# Autodesk Inventor assembly: minimal_frame_assembly
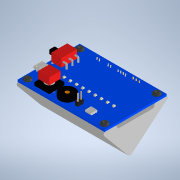
[picture p0: Inventor's stored thumbnail of the model, 180x180]
Saved by Autodesk Inventor 2020 (Build 240168000, 168)
## iProperties
Created: 2020-07-05
Part Number: minimal_frame_assembly
Document SubType Name: Assembly
Designer: Lukasz
Author: Lukasz
## Documents named in this file (7)
- C:\LUKE\PROJECTS\POMODORO\Mechanical\Assemblies\minimal_frame_assembly.iam
- C:\LUKE\PROJECTS\POMODORO\Mechanical\Assemblies\Board\Board_Pomodoro_v1.0.iam
- C:\LUKE\PROJECTS\POMODORO\Mechanical\Parts\minimal_frame_right.ipt
- C:\LUKE\PROJECTS\POMODORO\Mechanical\Parts\Standard\knurled_insert_M3_4.ipt
- C:\LUKE\PROJECTS\POMODORO\Mechanical\Parts\Standard\BATTERY_1S_560MAH_AKYGA.ipt
- C:\Users\Lukasz\Documents\Inventor\Content Center Files\R2020\en-US\ISO 7380-1\ISO 7380-1 - M3 x 6.ipt
- C:\LUKE\PROJECTS\POMODORO\Mechanical\Parts\battery_mount_1s_500mah.ipt
## Components (10 placed, 6 different names)
1. Board_Pomodoro_v1.0:1 [sub-assembly] — Rotational:1, Rotational:2, Flush:1, Angle:1, Rigid:3, Rigid:4, Rigid:5, Rigid:6
2. minimal_frame_right:1 — Rotational:1, Rotational:2, Rigid:1, Rigid:2, Mate:1, Cylindrical:1, Cylindrical:2
3. knurled_insert_M3_4:1 — Rigid:2
4. knurled_insert_M3_4:2 — Rigid:1
5. BATTERY_1S_560MAH_AKYGA:1 — Flush:1, Angle:1, Mate:1, Mate:2, Mate:3
6. ISO 7380-1 M3 x 6:1 — Rigid:3
7. ISO 7380-1 M3 x 6:2 — Rigid:6
8. ISO 7380-1 M3 x 6:3 — Rigid:4
9. ISO 7380-1 M3 x 6:4 — Rigid:5
10. battery_mount_1s_500mah:2 — Mate:2, Mate:3, Cylindrical:1, Cylindrical:2
## Relationships (15: WeldJoint 6, Mate 3, RevoluteJoint 2, CylindricalJoint 2, Flush 1, Angle 1)
- Rotational:1 [RevoluteJoint]: Board_Pomodoro_v1.0:1 ↔ minimal_frame_right:1
- Rotational:2 [RevoluteJoint]: Board_Pomodoro_v1.0:1 ↔ minimal_frame_right:1
- Rigid:1 [WeldJoint]: minimal_frame_right:1 ↔ knurled_insert_M3_4:2
- Rigid:2 [WeldJoint]: minimal_frame_right:1 ↔ knurled_insert_M3_4:1
- Flush:1 (-10 mm): Board_Pomodoro_v1.0:1 ↔ BATTERY_1S_560MAH_AKYGA:1
- Angle:1 (180 deg): Board_Pomodoro_v1.0:1 ↔ BATTERY_1S_560MAH_AKYGA:1
- Rigid:3 [WeldJoint]: Board_Pomodoro_v1.0:1 ↔ ISO 7380-1 M3 x 6:1
- Rigid:4 [WeldJoint]: Board_Pomodoro_v1.0:1 ↔ ISO 7380-1 M3 x 6:3
- Rigid:5 [WeldJoint]: Board_Pomodoro_v1.0:1 ↔ ISO 7380-1 M3 x 6:4
- Rigid:6 [WeldJoint]: Board_Pomodoro_v1.0:1 ↔ ISO 7380-1 M3 x 6:2
- Mate:1 (0.5 mm): minimal_frame_right:1 ↔ BATTERY_1S_560MAH_AKYGA:1
- Mate:2: BATTERY_1S_560MAH_AKYGA:1 ↔ battery_mount_1s_500mah:2
- Mate:3: BATTERY_1S_560MAH_AKYGA:1 ↔ battery_mount_1s_500mah:2
- Cylindrical:1: minimal_frame_right:1 ↔ battery_mount_1s_500mah:2
- Cylindrical:2: minimal_frame_right:1 ↔ battery_mount_1s_500mah:2
